# Autodesk Inventor assembly: warehouse
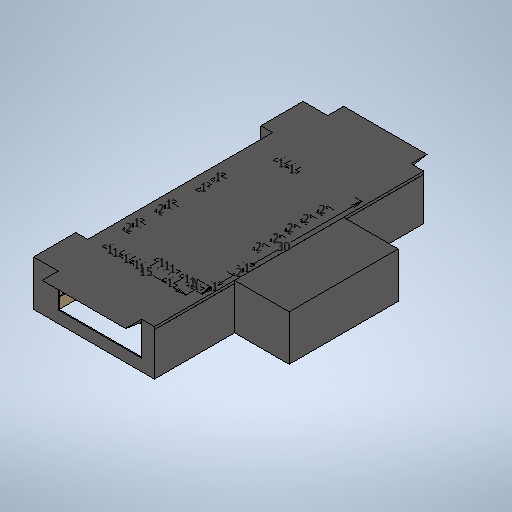
[picture p0: Inventor's stored thumbnail of the model, 512x512]
Saved by Autodesk Inventor 2025 (Build 290162000, 162)
## iProperties
Created: 2025-03-04
Part Number: warehouse
Document SubType Name: Assembly
Designer: Ennis
Author: Ennis
## Documents named in this file (3)
- C:\Users\ennis\Documents\Financien_Werk_OV\my_works\Courses TM\2024-2025\Semester 2\Practise Entreprise\warehouse\warehouse.iam
- C:\Users\ennis\Documents\Financien_Werk_OV\my_works\Courses TM\2024-2025\Semester 2\Practise Entreprise\warehouse\warehouse_base.ipt
- C:\Users\ennis\Documents\Financien_Werk_OV\my_works\Courses TM\2024-2025\Semester 2\Practise Entreprise\JetRacer\3D_Model_step\warehouse_reck.ipt
## Components (7 placed, 2 different names)
1. warehouse_base:1 — Flush:1
2. warehouse_reck:1 — Flush:1
3. warehouse_reck:2
4. warehouse_reck:3
5. warehouse_reck:4
6. warehouse_reck:5
7. warehouse_reck:6
## Relationships (1: Flush 1)
- Flush:1: warehouse_base:1 ↔ warehouse_reck:1
